# Autodesk Inventor assembly: 조립품1
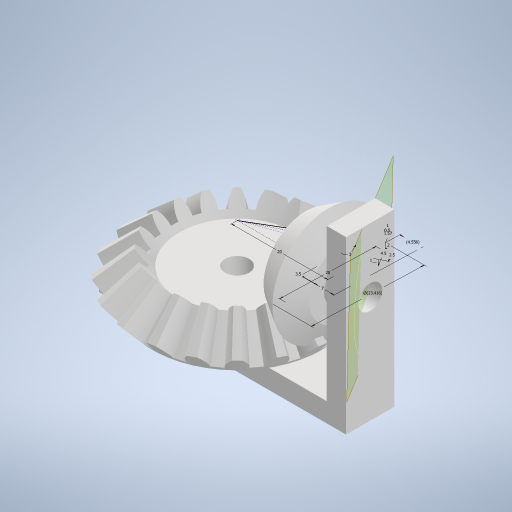
[picture p0: Inventor's stored thumbnail of the model, 512x512]
Saved by Autodesk Inventor 2023 (Build 270158000, 158)
## iProperties
Created: 2022-06-18
Part Number: 조립품1
Document SubType Name: Assembly
Designer: fly01
Author: fly01
## Documents named in this file (4)
- C:\Users\fly01\Desktop\베이맥스\설계\설계 테스트\조립품1.iam
- C:\Users\fly01\Desktop\베이맥스\설계\설계 테스트\베벨기어 001.ipt
- C:\Users\fly01\Desktop\베이맥스\설계\설계 테스트\베벨기어 002.ipt
- C:\Users\fly01\Desktop\베이맥스\설계\설계 테스트\베벨기어 003.ipt
## Components (3 placed, 3 different names)
1. 베벨기어 001:1 — 삽입:1
2. 베벨기어 002:1 — 삽입:2
3. 베벨기어 003:1 — 삽입:1, 삽입:2
## Relationships (2: Insert 2)
- 삽입:1 [Insert]: 베벨기어 001:1 ↔ 베벨기어 003:1
- 삽입:2 [Insert]: 베벨기어 002:1 ↔ 베벨기어 003:1
